# Autodesk Inventor assembly: cartesian_arm
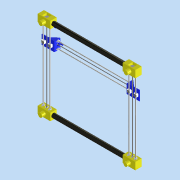
[picture p0: Inventor's stored thumbnail of the model, 180x180]
Saved by Autodesk Inventor 2022 (Build 260153000, 153)
## iProperties
Created: 2021-04-24
Part Number: cartesian_arm
Document SubType Name: Assembly
Designer: nnico
Author: nnico
## Documents named in this file (16)
- C:\Users\nnico\Documents\Desminado Humanitario\Repositories\gpr20_cartesian_arm\assemblies\cartesian_arm.iam
- C:\Users\nnico\Documents\Desminado Humanitario\Repositories\gpr20_cartesian_arm\ipt\x_axis_driver.ipt
- C:\Users\nnico\Documents\Desminado Humanitario\Repositories\gpr20_cartesian_arm\ipt\left_axis_aux.ipt
- C:\Users\nnico\Documents\Desminado Humanitario\Repositories\gpr20_cartesian_arm\ipt\left_axis_driver.ipt
- C:\Users\nnico\Documents\Desminado Humanitario\Repositories\gpr20_cartesian_arm\assemblies\misc\SHF12.ipt
- C:\Users\nnico\Documents\Desminado Humanitario\Repositories\gpr20_cartesian_arm\assemblies\misc\NEMA23_MOTOR.ipt
- C:\Users\nnico\Documents\Desminado Humanitario\Repositories\gpr20_cartesian_arm\assemblies\misc\12MM_1000MM_ROD.ipt
- C:\Users\nnico\Documents\Desminado Humanitario\Repositories\gpr20_cartesian_arm\assemblies\misc\SC12UU.ipt
- C:\Users\nnico\Documents\Desminado Humanitario\Repositories\gpr20_cartesian_arm\assemblies\misc\KFL08.ipt
- C:\Users\nnico\Documents\Desminado Humanitario\Repositories\gpr20_cartesian_arm\assemblies\misc\2inx100cm_pipe.ipt
- C:\Users\nnico\Documents\Desminado Humanitario\Repositories\gpr20_cartesian_arm\ipt\right_axis_driver.ipt
- C:\Users\nnico\Documents\Desminado Humanitario\Repositories\gpr20_cartesian_arm\ipt\right_axis_aux.ipt
- C:\Users\nnico\Documents\Desminado Humanitario\Repositories\gpr20_cartesian_arm\ipt\x_axis_aux.ipt
- C:\Users\nnico\Documents\Desminado Humanitario\Repositories\gpr20_cartesian_arm\assemblies\misc\8MM_1000MM_SCREW.ipt
- C:\Users\nnico\Documents\Desminado Humanitario\Repositories\gpr20_cartesian_arm\ipt\y_extender.ipt
- C:\Users\nnico\Documents\Desminado Humanitario\Repositories\gpr20_cartesian_arm\ipt\x_extender.ipt
## Components (41 placed, 15 different names)
1. x_axis_driver:1 — Rotational:4, Rotational:5, Rigid:10, Rigid:11, Rigid:12, Rigid:26
2. left_axis_aux:1 — Rigid:7, Rigid:8, Rigid:9, Rigid:13
3. left_axis_driver:1 — Flush:1, Mate:1, Mate:2, Rigid:1, Rigid:2, Rotational:1, Rotational:8, Rigid:27
4. SHF12:1 — Rigid:1, Rigid:3
5. SHF12:2 — Rigid:2, Rigid:4
6. NEMA23_MOTOR:1 — Rotational:1
7. 12MM_1000MM_ROD:1 — Rigid:3, Mate:3, Rotational:2
8. 12MM_1000MM_ROD:2 — Rigid:4, Mate:4, Rotational:3
9. SC12UU:1 — Mate:3, Rotational:4
10. SC12UU:2 — Mate:4, Rotational:5
11. SHF12:3 — Rigid:7, Rotational:3
12. SHF12:4 — Rigid:10, Rotational:7
13. KFL08:1 — Rigid:9, Rotational:16
14. SHF12:5 — Rigid:11, Rotational:6
15. SHF12:6 — Rigid:8, Rotational:2
16. 12MM_1000MM_ROD:3 — Rotational:6
17. 12MM_1000MM_ROD:4 — Rotational:7, Rotational:14
18. NEMA23_MOTOR:2 — Rigid:12
19. 2inx100cm_pipe:1 — Rotational:8, Rotational:9
20. 2inx100cm_pipe:2 — Rigid:13, Rotational:10
21. right_axis_driver:1 — Rotational:9, Rigid:16, Rigid:17, Rigid:19
22. right_axis_aux:1 — Rotational:10, Rigid:14, Rigid:15, Rigid:18
23. SHF12:7 — Rigid:16, Rotational:12
24. SHF12:8 — Rigid:17, Rotational:11
25. SHF12:9 — Rigid:14, Rotational:13
26. SHF12:10 — Rigid:15
27. NEMA23_MOTOR:3 — Rigid:19
28. KFL08:2 — Rigid:18, Rotational:15
29. 12MM_1000MM_ROD:5 — Rotational:12, Mate:5
30. 12MM_1000MM_ROD:6 — Rotational:11, Rotational:13, Mate:6
31. SC12UU:3 — Mate:5, Rigid:20
32. SC12UU:4 — Mate:6, Rigid:21
33. x_axis_aux:1 — Rigid:20, Rigid:21, Rigid:22, Rigid:23, Rigid:24
34. SHF12:11 — Rigid:22, Rotational:14
35. SHF12:12 — Rigid:23
36. KFL08:3 — Rigid:24, Rotational:17
37. 8MM_1000MM_SCREW:1 — Rotational:17
38. 8MM_1000MM_SCREW:2 — Rotational:15
39. 8MM_1000MM_SCREW:3 — Rotational:16
40. x_extender:1 — Rigid:26
41. y_extender:1 — Rigid:27
## Relationships (48: WeldJoint 24, RevoluteJoint 17, Mate 6, Flush 1)
- Flush:1: left_axis_driver:1
- Mate:1: left_axis_driver:1
- Mate:2: left_axis_driver:1
- Rigid:1 [WeldJoint]: left_axis_driver:1 ↔ SHF12:1
- Rigid:2 [WeldJoint]: left_axis_driver:1 ↔ SHF12:2
- Rotational:1 [RevoluteJoint]: left_axis_driver:1 ↔ NEMA23_MOTOR:1
- Rigid:3 [WeldJoint]: SHF12:1 ↔ 12MM_1000MM_ROD:1
- Rigid:4 [WeldJoint]: SHF12:2 ↔ 12MM_1000MM_ROD:2
- Mate:3: 12MM_1000MM_ROD:1 ↔ SC12UU:1
- Mate:4: 12MM_1000MM_ROD:2 ↔ SC12UU:2
- Rigid:7 [WeldJoint]: left_axis_aux:1 ↔ SHF12:3
- Rigid:8 [WeldJoint]: left_axis_aux:1 ↔ SHF12:6
- Rigid:9 [WeldJoint]: left_axis_aux:1 ↔ KFL08:1
- Rotational:2 [RevoluteJoint]: 12MM_1000MM_ROD:1 ↔ SHF12:6
- Rotational:3 [RevoluteJoint]: 12MM_1000MM_ROD:2 ↔ SHF12:3
- Rotational:4 [RevoluteJoint]: x_axis_driver:1 ↔ SC12UU:1
- Rotational:5 [RevoluteJoint]: x_axis_driver:1 ↔ SC12UU:2
- Rigid:10 [WeldJoint]: x_axis_driver:1 ↔ SHF12:4
- Rigid:11 [WeldJoint]: x_axis_driver:1 ↔ SHF12:5
- Rotational:6 [RevoluteJoint]: SHF12:5 ↔ 12MM_1000MM_ROD:3
- Rotational:7 [RevoluteJoint]: SHF12:4 ↔ 12MM_1000MM_ROD:4
- Rigid:12 [WeldJoint]: x_axis_driver:1 ↔ NEMA23_MOTOR:2
- Rotational:8 [RevoluteJoint]: left_axis_driver:1 ↔ 2inx100cm_pipe:1
- Rigid:13 [WeldJoint]: left_axis_aux:1 ↔ 2inx100cm_pipe:2
- Rotational:9 [RevoluteJoint]: 2inx100cm_pipe:1 ↔ right_axis_driver:1
- Rotational:10 [RevoluteJoint]: 2inx100cm_pipe:2 ↔ right_axis_aux:1
- Rigid:14 [WeldJoint]: right_axis_aux:1 ↔ SHF12:9
- Rigid:15 [WeldJoint]: right_axis_aux:1 ↔ SHF12:10
- Rigid:16 [WeldJoint]: right_axis_driver:1 ↔ SHF12:7
- Rigid:17 [WeldJoint]: right_axis_driver:1 ↔ SHF12:8
- Rigid:18 [WeldJoint]: right_axis_aux:1 ↔ KFL08:2
- Rigid:19 [WeldJoint]: right_axis_driver:1 ↔ NEMA23_MOTOR:3
- Rotational:11 [RevoluteJoint]: SHF12:8 ↔ 12MM_1000MM_ROD:6
- Rotational:12 [RevoluteJoint]: SHF12:7 ↔ 12MM_1000MM_ROD:5
- Rotational:13 [RevoluteJoint]: SHF12:9 ↔ 12MM_1000MM_ROD:6
- Mate:5: 12MM_1000MM_ROD:5 ↔ SC12UU:3
- Mate:6: 12MM_1000MM_ROD:6 ↔ SC12UU:4
- Rigid:20 [WeldJoint]: SC12UU:3 ↔ x_axis_aux:1
- Rigid:21 [WeldJoint]: SC12UU:4 ↔ x_axis_aux:1
- Rigid:22 [WeldJoint]: x_axis_aux:1 ↔ SHF12:11
- Rigid:23 [WeldJoint]: x_axis_aux:1 ↔ SHF12:12
- Rotational:14 [RevoluteJoint]: 12MM_1000MM_ROD:4 ↔ SHF12:11
- Rigid:24 [WeldJoint]: x_axis_aux:1 ↔ KFL08:3
- Rotational:15 [RevoluteJoint]: KFL08:2 ↔ 8MM_1000MM_SCREW:2
- Rotational:16 [RevoluteJoint]: KFL08:1 ↔ 8MM_1000MM_SCREW:3
- Rotational:17 [RevoluteJoint]: KFL08:3 ↔ 8MM_1000MM_SCREW:1
- Rigid:26 [WeldJoint]: x_axis_driver:1 ↔ x_extender:1
- Rigid:27 [WeldJoint]: left_axis_driver:1 ↔ y_extender:1
